# Autodesk Inventor assembly: SansRotor
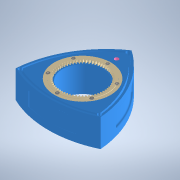
[picture p0: Inventor's stored thumbnail of the model, 180x180]
Saved by Autodesk Inventor 2022 (Build 260153000, 153)
## iProperties
Created: 2022-04-12
Part Number: SansRotor
Document SubType Name: Assembly
Designer: Janina
Author: Janina
## Documents named in this file (4)
- C:\Users\Janina\Desktop\CoceiJ\7 - Wankel\SansRotor.iam
- C:\Users\Janina\Desktop\CoceiJ\7 - Wankel\Rotor.ipt
- C:\Users\Janina\Desktop\CoceiJ\7 - Wankel\Roata.ipt
- D:\My Documents\Inventor\Content Center Files\R2022\en-US\ISO 4762(1)\DIN EN ISO 4762 - M4 x 6.ipt
## Components (8 placed, 3 different names)
1. Rotor:1 — Mate:1, Mate:2, Mate:3, Mate:4, Mate:5, Angle:1
2. Roata:1 — Mate:4, Mate:5, Angle:1, Insert:1, Insert:2, Insert:3, Insert:4, Insert:5, Insert:6
3. DIN EN ISO 4762 M4 x 6:1 — Insert:1
4. DIN EN ISO 4762 M4 x 6:2 — Insert:2
5. DIN EN ISO 4762 M4 x 6:3 — Insert:3
6. DIN EN ISO 4762 M4 x 6:4 — Insert:4
7. DIN EN ISO 4762 M4 x 6:5 — Insert:5
8. DIN EN ISO 4762 M4 x 6:6 — Insert:6
## Relationships (12: Insert 6, Mate 5, Angle 1)
- Mate:1: Rotor:1
- Mate:2: Rotor:1
- Mate:3: Rotor:1
- Mate:4: Rotor:1 ↔ Roata:1
- Mate:5: Rotor:1 ↔ Roata:1
- Angle:1 (0 deg): Rotor:1 ↔ Roata:1
- Insert:1: Roata:1 ↔ DIN EN ISO 4762 M4 x 6:1
- Insert:2: Roata:1 ↔ DIN EN ISO 4762 M4 x 6:2
- Insert:3: Roata:1 ↔ DIN EN ISO 4762 M4 x 6:3
- Insert:4: Roata:1 ↔ DIN EN ISO 4762 M4 x 6:4
- Insert:5: Roata:1 ↔ DIN EN ISO 4762 M4 x 6:5
- Insert:6: Roata:1 ↔ DIN EN ISO 4762 M4 x 6:6
